# Autodesk Inventor assembly: Motor_with_wheel
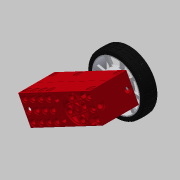
[picture p0: Inventor's stored thumbnail of the model, 180x180]
Saved by Autodesk Inventor 2019.3 (Build 233278000, 278)
## iProperties
Created: 2019-03-18
Part Number: Motor_with_wheel
Document SubType Name: Assembly
Designer: Varga Daniel
Author: Varga Daniel
## Documents named in this file (4)
- C:\!_Dani\!_cloud\OneDrive\!_munka\Revolution\RevvyDemoKit\Structural parts\Test assemblies\Motor_with_wheel_conn_side.iam
- C:\!_Dani\!_cloud\OneDrive\!_munka\Revolution\RevvyDemoKit\Structural parts\Demo parts\Wheel\Inventor imported\wheel_tyre.iam
- C:\!_Dani\!_cloud\OneDrive\!_munka\Revolution\RevvyDemoKit\Structural parts\Demo parts\Motor\Inventor imported\motor.iam
- C:\!_Dani\!_cloud\OneDrive\!_munka\Revolution\RevvyDemoKit\Structural parts\Connetor Pins\CP1+x1+\CP1x1.ipt
## Components (6 placed, 3 different names)
1. wheel_tyre:1 [sub-assembly] — Insert:5, Insert:6
2. motor:1 [sub-assembly] — Insert:1, Insert:2, Insert:3, Insert:4
3. CP1x1:1 — Insert:2
4. CP1x1:2 — Insert:1, Insert:5
5. CP1x1:3 — Insert:4
6. CP1x1:4 — Insert:3, Insert:6
## Relationships (6: Insert 6)
- Insert:1: motor:1 ↔ CP1x1:2
- Insert:2: motor:1 ↔ CP1x1:1
- Insert:3: motor:1 ↔ CP1x1:4
- Insert:4: motor:1 ↔ CP1x1:3
- Insert:5: wheel_tyre:1 ↔ CP1x1:2
- Insert:6: wheel_tyre:1 ↔ CP1x1:4
